# Autodesk Inventor assembly: smart locker final
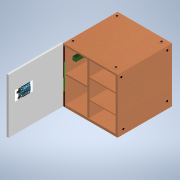
[picture p0: Inventor's stored thumbnail of the model, 180x180]
Saved by Autodesk Inventor 2022 (Build 260153000, 153)
## iProperties
Created: 2021-07-10
Part Number: smart locker final
Document SubType Name: Assembly
Designer: Hp
Author: Hp
## Documents named in this file (6)
- F:\final locker\smart locker final.iam
- F:\final locker\locker 2.ipt
- F:\final locker\Part3.ipt
- F:\final locker\lock4.ipt
- F:\final locker\Rack and Pinion-Drive.iam
- F:\final locker\lock1.ipt
## Components (26 placed, 5 different names)
1. locker 2:1 — Mate:1, Angle:1, Mate:2, Mate:4, Mate:5, Mate:6, Mate:7, Mate:8, Mate:9, Mate:10, Mate:11, Mate:12, Mate:13, Mate:14, Mate:15, Mate:16, Mate:17, Mate:18, Mate:19, Mate:20, Mate:21, Mate:22, Mate:23, Mate:24, Mate:25
2. Part3:1 — Mate:1, Angle:1, Mate:3
3. lock4:1 — Mate:2
4. lock4:2 — Mate:3
5. lock4:3 — Mate:4
6. Rack and Pinion-Drive:1 [sub-assembly] — Mate:5
7. lock1:1 — Mate:12
8. lock1:2 — Mate:6
9. lock1:3 — Mate:11
10. lock1:4 — Mate:21
11. lock1:5 — Mate:18
12. lock1:6 — Mate:13
13. lock1:7 — Mate:9
14. lock1:8 — Mate:10
15. lock1:9 — Mate:7
16. lock1:10 — Mate:23
17. lock1:11 — Mate:25
18. lock1:12 — Mate:8
19. lock1:13 — Mate:24
20. lock1:14 — Mate:17
21. lock1:15 — Mate:19
22. lock1:16 — Mate:15
23. lock1:17 — Mate:14
24. lock1:18 — Mate:16
25. lock1:19 — Mate:20
26. lock1:20 — Mate:22
## Relationships (26: Mate 25, Angle 1)
- Mate:1: locker 2:1 ↔ Part3:1
- Angle:1 (-90 deg): locker 2:1 ↔ Part3:1
- Mate:2: locker 2:1 ↔ lock4:1
- Mate:3: Part3:1 ↔ lock4:2
- Mate:4: locker 2:1 ↔ lock4:3
- Mate:5: locker 2:1 ↔ Rack and Pinion-Drive:1
- Mate:6: locker 2:1 ↔ lock1:2
- Mate:7: locker 2:1 ↔ lock1:9
- Mate:8: locker 2:1 ↔ lock1:12
- Mate:9: locker 2:1 ↔ lock1:7
- Mate:10: locker 2:1 ↔ lock1:8
- Mate:11: locker 2:1 ↔ lock1:3
- Mate:12: locker 2:1 ↔ lock1:1
- Mate:13: locker 2:1 ↔ lock1:6
- Mate:14: locker 2:1 ↔ lock1:17
- Mate:15: locker 2:1 ↔ lock1:16
- Mate:16: locker 2:1 ↔ lock1:18
- Mate:17: locker 2:1 ↔ lock1:14
- Mate:18: locker 2:1 ↔ lock1:5
- Mate:19: locker 2:1 ↔ lock1:15
- Mate:20: locker 2:1 ↔ lock1:19
- Mate:21: locker 2:1 ↔ lock1:4
- Mate:22: locker 2:1 ↔ lock1:20
- Mate:23: locker 2:1 ↔ lock1:10
- Mate:24: locker 2:1 ↔ lock1:13
- Mate:25: locker 2:1 ↔ lock1:11
